# Autodesk Inventor assembly: SPM
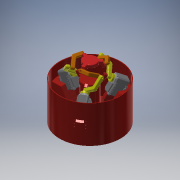
[picture p0: Inventor's stored thumbnail of the model, 180x180]
Saved by Autodesk Inventor 2019 (Build 230136000, 136)
## iProperties
Created: 2022-07-14
Part Number: SPM
Document SubType Name: Assembly
Designer: zreik
Author: zreik
## Documents named in this file (6)
- D:\Documents\HIAST\4th year\4th Year Project\Design\SPM.iam
- D:\Documents\HIAST\4th year\4th Year Project\Design\BottomPlatform.ipt
- D:\Documents\HIAST\4th year\4th Year Project\Design\TopPlatform.ipt
- D:\Documents\HIAST\4th year\4th Year Project\Design\Link1.ipt
- D:\Documents\HIAST\4th year\4th Year Project\Design\Link2.ipt
- D:\Documents\HIAST\4th year\4th Year Project\Design\AX-12A\AX-12A.iam
## Components (11 placed, 5 different names)
1. BottomPlatform:1 — Mate:3, Mate:11, Mate:12, Mate:13, Angle:1, Angle:2, Mate:34, Mate:37, Mate:38, Mate:39
2. TopPlatform:1 — Mate:7, Mate:8, Mate:9, Mate:10, Angle:1, Mate:30, Mate:32, Mate:36
3. Link1:1 — Mate:3, Mate:5, Mate:40
4. Link2:1 — Mate:5, Mate:7, Mate:30
5. Link1:2 — Mate:33, Mate:34
6. Link2:2 — Mate:32, Mate:33
7. Link1:3 — Mate:35, Mate:37
8. Link2:3 — Mate:35, Mate:36
9. AX-12A:1 [sub-assembly] — Mate:38, Mate:39, Mate:40
10. AX-12A:2 [sub-assembly]
11. AX-12A:3 [sub-assembly]
## Component patterns: (3 elements, first: AX-12A:1)
## Relationships (27: Mate 25, Angle 2)
- Mate:3: BottomPlatform:1 ↔ Link1:1
- Mate:5: Link1:1 ↔ Link2:1
- Mate:7: TopPlatform:1 ↔ Link2:1
- Mate:8: TopPlatform:1
- Mate:9: TopPlatform:1
- Mate:10: TopPlatform:1
- Mate:11: BottomPlatform:1
- Mate:12: BottomPlatform:1
- Mate:13: BottomPlatform:1
- Mate:14
- Mate:15
- Mate:16
- Mate:17
- Mate:27
- Angle:1 (0 deg): BottomPlatform:1 ↔ TopPlatform:1
- Mate:30: TopPlatform:1 ↔ Link2:1
- Mate:31
- Angle:2 (0 deg): BottomPlatform:1
- Mate:32: TopPlatform:1 ↔ Link2:2
- Mate:33: Link1:2 ↔ Link2:2
- Mate:34: BottomPlatform:1 ↔ Link1:2
- Mate:35: Link1:3 ↔ Link2:3
- Mate:36: TopPlatform:1 ↔ Link2:3
- Mate:37: BottomPlatform:1 ↔ Link1:3
- Mate:38: BottomPlatform:1 ↔ AX-12A:1
- Mate:39: BottomPlatform:1 ↔ AX-12A:1
- Mate:40: Link1:1 ↔ AX-12A:1
